# Autodesk Inventor assembly: DiaD bumper fastener subassy
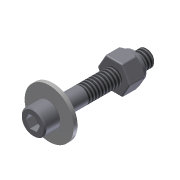
[picture p0: Inventor's stored thumbnail of the model, 180x180]
Saved by Autodesk Inventor 2013 (Build 170138000, 138)
## iProperties
Created: 2013-05-20
Part Number: DiaD bumper fastener subassy
Document SubType Name: Assembly
Designer: Nemo
Author: Nemo
## Documents named in this file (4)
- H:\Nemo\Documents\Robotics\COTS Parts\Drive in a Day\DiaD bumper fastener subassy.iam
- H:\Nemo\Documents\Robotics\COTS Parts\Fasteners\14-20 locknut.ipt
- H:\Nemo\Documents\Robotics\COTS Parts\Fasteners\14-20 SHCS x1500.ipt
- H:\Nemo\Documents\Robotics\COTS Parts\Fasteners\14-20 Washer - Flat.ipt
## Components (3 placed, 3 different names)
1. 14-20 locknut:1
2. 14-20 SHCS x1500:1
3. 14-20 Washer - Flat:1
## Relationships (3: Insert 1, Mate 1, Flush 1)
- [Insert]: 14-20 SHCS x1500:1 ↔ 14-20 Washer - Flat:1
- [Mate]: 14-20 locknut:1 ↔ 14-20 SHCS x1500:1
- [Flush] (5.08 mm): 14-20 locknut:1 ↔ 14-20 SHCS x1500:1
